# Autodesk Inventor assembly: Assembly13 (Cam hosuing sub )
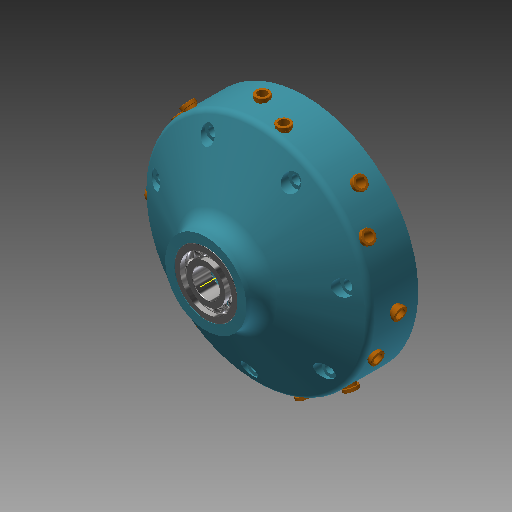
[picture p0: Inventor's stored thumbnail of the model, 512x512]
Saved by Autodesk Inventor 2018 (Build 220112000, 112)
## iProperties
Created: 2023-05-20
Part Number: Assembly13 (Cam hosuing sub )
Document SubType Name: Assembly
Designer: Habib Mohamed
Author: Habib Mohamed
## Documents named in this file (4)
- D:\Inventor\My projects\Rotary Engine\Assembly\Assembly13 (Cam hosuing sub ).iam
- D:\Inventor\My projects\Rotary Engine\Drum (Cam Hosuing).ipt
- D:\Inventor\My projects\Rotary Engine\Component 5(Ram Bearing).ipt
- C:\Users\Habib Mohamed\Documents\Inventor\Content Center Files\R2018\en-US\DIN 625 - T1\DIN 625 T1 - 6001 - 12 x 28 x 8.ipt
## Components (16 placed, 3 different names)
1. Drum (Cam Hosuing):1 — Mate:1, Mate:2, Tangent:1, Tangent:2, Mate:3, Mate:4, Mate:5
2. DIN 625 - T1 6001 - 12 x 28 x 8:1 — Mate:4, Mate:5
3. Component 5(Ram Bearing):2 — Mate:2, Tangent:1
4. Component 5(Ram Bearing):1 — Mate:1, Tangent:2
5. Component 5(Ram Bearing):3
6. Component 5(Ram Bearing):4
7. Component 5(Ram Bearing):5
8. Component 5(Ram Bearing):6
9. Component 5(Ram Bearing):7
10. Component 5(Ram Bearing):8
11. Component 5(Ram Bearing):9
12. Component 5(Ram Bearing):10
13. Component 5(Ram Bearing):11
14. Component 5(Ram Bearing):12
15. Component 5(Ram Bearing):13
16. Component 5(Ram Bearing):14
## Component patterns: (7 elements, first: Component 5(Ram Bearing):2 + Component 5(Ram Bearing):1)
## Relationships (7: Mate 5, Tangent 2)
- Mate:1: Drum (Cam Hosuing):1 ↔ Component 5(Ram Bearing):1
- Mate:2: Drum (Cam Hosuing):1 ↔ Component 5(Ram Bearing):2
- Tangent:1: Drum (Cam Hosuing):1 ↔ Component 5(Ram Bearing):2
- Tangent:2: Drum (Cam Hosuing):1 ↔ Component 5(Ram Bearing):1
- Mate:3: Drum (Cam Hosuing):1
- Mate:4: Drum (Cam Hosuing):1 ↔ DIN 625 - T1 6001 - 12 x 28 x 8:1
- Mate:5: Drum (Cam Hosuing):1 ↔ DIN 625 - T1 6001 - 12 x 28 x 8:1
